# Autodesk Inventor assembly: JALTARANG_BOT
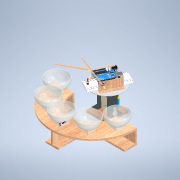
[picture p0: Inventor's stored thumbnail of the model, 180x180]
Saved by Autodesk Inventor 2021 (Build 250183000, 183)
## iProperties
Created: 2021-07-24
Part Number: JALTARANG_BOT
Document SubType Name: Assembly
Designer: KAVYA
Author: KAVYA
## Documents named in this file (20)
- H:\chiku\Musical_bot\JALTARANG_BOT.iam
- H:\chiku\Autodesk\Musical bot\Muisc_4\wc.ipt
- H:\chiku\Autodesk\Musical bot\Muisc_4\clamp.ipt
- H:\chiku\Autodesk\Musical bot\Muisc_4\base.ipt
- H:\chiku\Autodesk\Musical bot\Muisc_4\DONG CO 775.ipt
- H:\chiku\Autodesk\Musical bot\Music\Box.ipt
- H:\chiku\Autodesk\Musical bot\closing_plate.ipt
- H:\chiku\Autodesk\Musical bot\Muisc_4\Servo Motor SG90.0001.ipt
- H:\chiku\Autodesk\Musical bot\Muisc_4\horn.0001.ipt
- H:\chiku\Autodesk\Musical bot\Muisc_4\arm.ipt
- H:\chiku\Autodesk\Musical bot\Muisc_4\armscrew.ipt
- H:\chiku\Autodesk\Musical bot\Muisc_4\armscrew1.ipt
- H:\chiku\Autodesk\Musical bot\Muisc_4\Cuptable1.ipt
- H:\chiku\Autodesk\Musical bot\Muisc_4\screw m10x40.ipt
- H:\chiku\Autodesk\Musical bot\Muisc_4\nut m10.ipt
- H:\chiku\Autodesk\Musical bot\Muisc_4\Bowlcup.ipt
- H:\chiku\arduino-uno-micro-processor-1.snapshot.4\ardino.ipt
- H:\chiku\ELEctronic\protoboard.ipt
- H:\chiku\ELEctronic\Push Button.ipt
- H:\chiku\Autodesk\Shreya_music\Battery_updated.ipt
## Components (30 placed, 19 different names)
1. clamp:1 — Mate:1, Mate:2, Mate:3, Mate:4, Mate:5, Mate:25, Mate:27
2. base:1 — Mate:1, Mate:2, Mate:3, Mate:20, Mate:21, Mate:22, Mate:23, Mate:34
3. DONG CO 775:1 — Mate:4, Mate:5, Rigid:1
4. Box:1 — Rigid:1, Rigid:2
5. closing_plate:1 — Rigid:2, Rigid:3, Mate:33, Rigid:8
6. wc:1 — Rigid:3, Cylindrical:1, Mate:6, Mate:7, Mate:8, Mate:9, Mate:10, Mate:11, Mate:12, Mate:13, Rigid:7
7. Servo Motor SG90.0001:1 — Mate:10, Mate:11, Mate:12, Mate:13, Mate:14, Mate:15
8. Servo Motor SG90.0001:2 — Cylindrical:1, Mate:6, Mate:7, Mate:8, Mate:9, Mate:16, Mate:17
9. horn.0001:2 — Mate:14, Mate:15, Rotational:1, Rotational:4
10. horn.0001:3 — Mate:16, Mate:17, Rotational:2, Rotational:3
11. arm:1 — Rotational:1, Rigid:4, Mate:18, Mate:19, Rotational:4
12. arm:2 — Rotational:2, Rigid:5, Rotational:3, Rigid:6
13. armscrew:1 — Rigid:5
14. armscrew:2 — Rigid:4
15. armscrew1:1 — Rigid:6
16. armscrew1:2 — Mate:18, Mate:19
17. Cuptable1:1 — Mate:28, Mate:29, Mate:30, Mate:31, Mate:32
18. screw m10x40:1 — Mate:22, Mate:23, Mate:26
19. screw m10x40:2 — Mate:20, Mate:21, Mate:24
20. nut m10:1 — Mate:24, Mate:25
21. nut m10:2 — Mate:26, Mate:27
22. Bowlcup:1 — Mate:28
23. Bowlcup:2 — Mate:29
24. Bowlcup:3 — Mate:30
25. Bowlcup:4 — Mate:31
26. Bowlcup:5 — Mate:32
27. ardino:1 — Rigid:7
28. protoboard:1 — Mate:33, Rigid:8, Rigid:9
29. Push Button:1 — Rigid:9
30. Battery_updated:1 — Mate:34
## Relationships (48: Mate 34, WeldJoint 9, RevoluteJoint 4, CylindricalJoint 1)
- Mate:1: clamp:1 ↔ base:1
- Mate:2: clamp:1 ↔ base:1
- Mate:3: clamp:1 ↔ base:1
- Mate:4: clamp:1 ↔ DONG CO 775:1
- Mate:5: clamp:1 ↔ DONG CO 775:1
- Rigid:1 [WeldJoint]: DONG CO 775:1 ↔ Box:1
- Rigid:2 [WeldJoint]: Box:1 ↔ closing_plate:1
- Rigid:3 [WeldJoint] (40 mm): closing_plate:1 ↔ wc:1
- Cylindrical:1: wc:1 ↔ Servo Motor SG90.0001:2
- Mate:6: wc:1 ↔ Servo Motor SG90.0001:2
- Mate:7: wc:1 ↔ Servo Motor SG90.0001:2
- Mate:8: wc:1 ↔ Servo Motor SG90.0001:2
- Mate:9: wc:1 ↔ Servo Motor SG90.0001:2
- Mate:10: wc:1 ↔ Servo Motor SG90.0001:1
- Mate:11: wc:1 ↔ Servo Motor SG90.0001:1
- Mate:12: wc:1 ↔ Servo Motor SG90.0001:1
- Mate:13: wc:1 ↔ Servo Motor SG90.0001:1
- Mate:14: Servo Motor SG90.0001:1 ↔ horn.0001:2
- Mate:15: Servo Motor SG90.0001:1 ↔ horn.0001:2
- Mate:16: Servo Motor SG90.0001:2 ↔ horn.0001:3
- Mate:17: Servo Motor SG90.0001:2 ↔ horn.0001:3
- Rotational:1 [RevoluteJoint]: horn.0001:2 ↔ arm:1
- Rotational:2 [RevoluteJoint]: horn.0001:3 ↔ arm:2
- Rigid:4 [WeldJoint]: arm:1 ↔ armscrew:2
- Rigid:5 [WeldJoint]: arm:2 ↔ armscrew:1
- Mate:18: arm:1 ↔ armscrew1:2
- Mate:19: arm:1 ↔ armscrew1:2
- Rotational:3 [RevoluteJoint]: horn.0001:3 ↔ arm:2
- Rotational:4 [RevoluteJoint]: horn.0001:2 ↔ arm:1
- Rigid:6 [WeldJoint]: arm:2 ↔ armscrew1:1
- Mate:20: base:1 ↔ screw m10x40:2
- Mate:21: base:1 ↔ screw m10x40:2
- Mate:22: base:1 ↔ screw m10x40:1
- Mate:23: base:1 ↔ screw m10x40:1
- Mate:24: screw m10x40:2 ↔ nut m10:1
- Mate:25: clamp:1 ↔ nut m10:1
- Mate:26: screw m10x40:1 ↔ nut m10:2
- Mate:27: clamp:1 ↔ nut m10:2
- Mate:28: Cuptable1:1 ↔ Bowlcup:1
- Mate:29: Cuptable1:1 ↔ Bowlcup:2
- Mate:30: Cuptable1:1 ↔ Bowlcup:3
- Mate:31: Cuptable1:1 ↔ Bowlcup:4
- Mate:32: Cuptable1:1 ↔ Bowlcup:5
- Rigid:7 [WeldJoint]: wc:1 ↔ ardino:1
- Mate:33: closing_plate:1 ↔ protoboard:1
- Rigid:8 [WeldJoint]: closing_plate:1 ↔ protoboard:1
- Rigid:9 [WeldJoint]: protoboard:1 ↔ Push Button:1
- Mate:34: base:1 ↔ Battery_updated:1
